# Autodesk Inventor assembly: LED and Diffusor
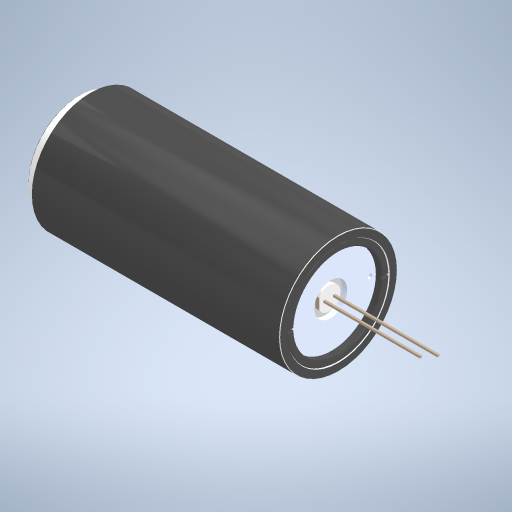
[picture p0: Inventor's stored thumbnail of the model, 512x512]
Saved by Autodesk Inventor 2023 (Build 270158030, 158C)
## iProperties
Created: 2025-06-04
Part Number: LED and Diffusor
Document SubType Name: Assembly
Designer: Julian
Author: Julian
## Documents named in this file (5)
- C:\Users\Julian\Desktop\backup_inventor and 3D-Print\inventor\LED reflection\LED and Diffusor.iam
- C:\Users\Julian\Desktop\backup_inventor and 3D-Print\inventor\LED reflection\SM1L25.ipt
- C:\Users\Julian\Desktop\backup_inventor and 3D-Print\inventor\LED reflection\DG10-600-A.ipt
- C:\Users\Julian\Desktop\backup_inventor and 3D-Print\inventor\LED reflection\S1LEDM.ipt
- C:\Users\Julian\Desktop\backup_inventor and 3D-Print\inventor\LED reflection\LEDW7E.ipt
## Components (4 placed, 4 different names)
1. SM1L25:1 — Passend:3, Fluchtend:1, Passend:4, Fluchtend:2
2. DG10-600-A:1 — Passend:4, Fluchtend:2
3. S1LEDM:1 — Passend:1, Passend:2, Passend:3, Fluchtend:1
4. LEDW7E:1 — Passend:1, Passend:2
## Relationships (6: Mate 4, Flush 2)
- Passend:1 [Mate]: S1LEDM:1 ↔ LEDW7E:1
- Passend:2 [Mate]: S1LEDM:1 ↔ LEDW7E:1
- Passend:3 [Mate]: SM1L25:1 ↔ S1LEDM:1
- Fluchtend:1 [Flush] (2 mm): SM1L25:1 ↔ S1LEDM:1
- Passend:4 [Mate]: SM1L25:1 ↔ DG10-600-A:1
- Fluchtend:2 [Flush] (4 mm): SM1L25:1 ↔ DG10-600-A:1
